# Autodesk Inventor assembly: RV24 v6
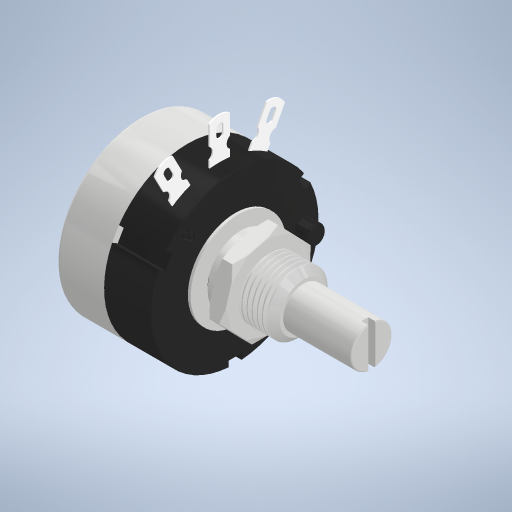
[picture p0: Inventor's stored thumbnail of the model, 512x512]
Saved by Autodesk Inventor 2024 (Build 280153000, 153)
## iProperties
Created: 2021-04-14
Part Number: RV24 v6
Document SubType Name: Assembly
Designer: ASUS
Sending System: Autodesk Translation Framework v10.6.0.1341
Preprocessor: ST-DEVELOPER v18.1
Title: C:/Users/frek2/Desktop/RV24 v6.step
## Documents named in this file (6)
- C:\Users\ASUS\Documents\Inventor\Tugas Akhir Stechoq\Assembly\RV24 v6.iam
- C:\Users\ASUS\Downloads\rv24yn-1.snapshot.5\RV24 v6\Shaft v3.ipt
- C:\Users\ASUS\Downloads\rv24yn-1.snapshot.5\RV24 v6\Body v5.ipt
- C:\Users\ASUS\Downloads\rv24yn-1.snapshot.5\RV24 v6\Puck M9 v2.ipt
- C:\Users\ASUS\Downloads\rv24yn-1.snapshot.5\RV24 v6\Engraver v3.ipt
- C:\Users\ASUS\Downloads\rv24yn-1.snapshot.5\RV24 v6\Nut M9 v2.ipt
## Components (5 placed, 5 different names)
1. Shaft v3:1 — Mate:5, Mate:6
2. Body v5:1 — Mate:3, Mate:4, Mate:5, Mate:6, Mate:7
3. Puck M9 v2:1 — Mate:1, Mate:2, Mate:3
4. Engraver v3:1 — Mate:1, Mate:2, Mate:4, Mate:8
5. Nut M9 v2:1 — Mate:7, Mate:8
## Relationships (8: Mate 8)
- Mate:1: Puck M9 v2:1 ↔ Engraver v3:1
- Mate:2: Puck M9 v2:1 ↔ Engraver v3:1
- Mate:3: Body v5:1 ↔ Puck M9 v2:1
- Mate:4: Body v5:1 ↔ Engraver v3:1
- Mate:5: Shaft v3:1 ↔ Body v5:1
- Mate:6: Shaft v3:1 ↔ Body v5:1
- Mate:7: Body v5:1 ↔ Nut M9 v2:1
- Mate:8: Engraver v3:1 ↔ Nut M9 v2:1
